# Autodesk Inventor assembly: Manipulator
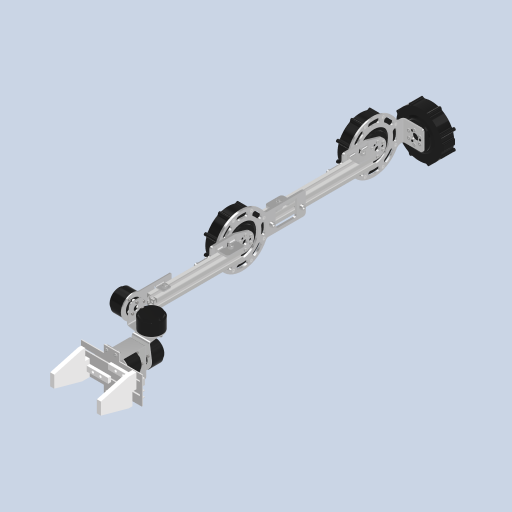
[picture p0: Inventor's stored thumbnail of the model, 512x512]
Saved by Autodesk Inventor 2023 (Build 270158000, 158)
## iProperties
Created: 2024-11-08
Part Number: Manipulator
Document SubType Name: Assembly
Designer: kiyo
Mass: 3708.17 g
Surface Area: 3992.73 cm^2
Volume: 794.407 cm^3
Density: 4.66785 g/cm^3
Author: kiyo
## Documents named in this file (21)
- D:\GitHub\inventor\syu-si\OfficeRobot\Manipulator\Manipulator.iam
- D:\GitHub\inventor\syu-si\OfficeRobot\ReadyMade\Steadywin\GIM8108-8.iam
- D:\GitHub\inventor\syu-si\OfficeRobot\ReadyMade\Steadywin\GIM3505-8_with-driver.ipt
- D:\GitHub\inventor\syu-si\OfficeRobot\Manipulator\wrist-pitch-plate.ipt
- D:\GitHub\inventor\syu-si\OfficeRobot\ReadyMade\Screw\M2-5_6mm.ipt
- D:\GitHub\inventor\syu-si\OfficeRobot\ReadyMade\Screw\CBSH3-8.ipt
- D:\GitHub\inventor\syu-si\OfficeRobot\ReadyMade\Screw\FWSJJ-D5-V2_6-T4_5.ipt
- D:\GitHub\inventor\syu-si\OfficeRobot\ReadyMade\Screw\M2-5_10mm.ipt
- D:\GitHub\inventor\syu-si\OfficeRobot\ReadyMade\Screw\HNTU5-5.ipt
- D:\GitHub\inventor\syu-si\OfficeRobot\Manipulator\sholder_roll_bracket.ipt
- D:\GitHub\inventor\syu-si\OfficeRobot\ReadyMade\Screw\SCB5-8.ipt
- D:\GitHub\inventor\syu-si\OfficeRobot\ReadyMade\Aluminum-frame\NFS5-2020-170-AV15-BV145.ipt
- D:\GitHub\inventor\syu-si\OfficeRobot\Manipulator\wrist_bracket.ipt
- D:\GitHub\inventor\syu-si\OfficeRobot\Hand\Hand.iam
- D:\GitHub\inventor\syu-si\OfficeRobot\ReadyMade\Screw\M2-5_9mm.ipt
- D:\GitHub\inventor\syu-si\OfficeRobot\Manipulator\pitch_plate.ipt
- D:\GitHub\inventor\syu-si\OfficeRobot\ReadyMade\Screw\SCB5-25.ipt
- D:\GitHub\inventor\syu-si\OfficeRobot\ReadyMade\Screw\SCB5-10.ipt
- D:\GitHub\inventor\syu-si\OfficeRobot\Manipulator\elbow-pitch-plate_T4.ipt
- D:\GitHub\inventor\syu-si\OfficeRobot\ReadyMade\Screw\HFBCM3-8.ipt
- D:\GitHub\inventor\syu-si\OfficeRobot\ReadyMade\Aluminum-frame\NFS5-2020-215-AV15-BV180.ipt
## Components (101 placed, 20 different names)
1. sholder_roll_bracket:1 — 挿入:350, 挿入:414, 挿入:493, 挿入:517, 挿入:526, 挿入:527, 挿入:528, 挿入:529, 挿入:530, 挿入:531, 挿入:532, 挿入:533, 挿入:534, 挿入:535, 挿入:536, 挿入:537, 挿入:538, 挿入:539
2. wrist_bracket:2 — 挿入:485, 挿入:552, 挿入:553, 挿入:554
3. wrist_bracket:1
4. wrist-pitch-plate:1 — メイト:71, メイト:72, 正接:48, 正接:49, 角度:76, 角度:77, 角度:78, 正接:50, 正接:51, 挿入:470, 挿入:471, 挿入:494, 挿入:495, 挿入:496
5. NFS5-2020-215-AV15-BV180:1
6. HNTU5-5:32 — 挿入:516
7. SCB5-25:3 — 挿入:516, 正接:83
8. HNTU5-5:33
9. SCB5-10:6 — 正接:84
10. HNTU5-5:34
11. SCB5-10:5 — 正接:85
12. NFS5-2020-170-AV15-BV145:1 — メイト:106, メイト:107, 角度:90, 角度:91, 正接:70, 正接:71, 角度:92, メイト:108, 正接:74, 正接:75, メイト:114, メイト:115
13. M2-5_6mm:16 — 挿入:494
14. M2-5_6mm:17 — 挿入:496
15. M2-5_6mm:18 — 挿入:495
16. Hand:1 [sub-assembly] — 挿入:497, 挿入:501, 挿入:502, 挿入:503, 角度:98, 角度:99
17. M2-5_9mm:1 — 挿入:498, 挿入:503
18. M2-5_9mm:2 — 挿入:500, 挿入:502
19. M2-5_9mm:3 — 挿入:499, 挿入:501
20. HNTU5-5:38
21. SCB5-25:1 — 正接:78
22. HNTU5-5:39
23. SCB5-10:1 — 正接:80
24. HNTU5-5:40
25. SCB5-10:2 — 正接:79
26. HNTU5-5:41 — 角度:90
27. SCB5-10:3 — メイト:106, 正接:70, 正接:82
28. HNTU5-5:42 — 角度:91
29. SCB5-10:4 — メイト:107, 正接:71, 正接:81
30. HNTU5-5:43 — 角度:92
31. SCB5-25:2 — メイト:108, 正接:74, 正接:75, 正接:77
32. pitch_plate:1 — 挿入:512, 正接:78, 正接:79, 正接:80, 角度:96, 挿入:540, 挿入:541, 挿入:542, 挿入:543, 挿入:544, 挿入:545
33. pitch_plate:2 — 挿入:513, メイト:114, メイト:115, 正接:77, 正接:81, 正接:82, 角度:97, 挿入:546, 挿入:547, 挿入:548, 挿入:549, 挿入:550, 挿入:551
34. elbow-pitch-plate_T4:1 — 挿入:514, 挿入:515, 正接:83, 挿入:518, 挿入:519, 挿入:520, 挿入:521, 挿入:522, 挿入:523, 挿入:524, 挿入:525, 正接:84, 正接:85
35. HFBCM3-8:1 — 挿入:521
36. HFBCM3-8:2 — 挿入:524
37. HFBCM3-8:3 — 挿入:525
38. HFBCM3-8:4 — 挿入:523
39. HFBCM3-8:5 — 挿入:522
40. HFBCM3-8:6 — 挿入:518
41. HFBCM3-8:7 — 挿入:519
42. HFBCM3-8:8 — 挿入:520
43. HFBCM3-8:9 — 挿入:531
44. HFBCM3-8:10 — 挿入:532
45. HFBCM3-8:11 — 挿入:530
46. HFBCM3-8:12 — 挿入:529
47. HFBCM3-8:13 — 挿入:528
48. HFBCM3-8:14 — 挿入:533
49. HFBCM3-8:15 — 挿入:526
50. HFBCM3-8:16 — 挿入:527
51. CBSH3-8:1 — 挿入:535
52. CBSH3-8:2 — 挿入:536
53. CBSH3-8:3 — 挿入:538
54. CBSH3-8:4 — 挿入:539
55. CBSH3-8:5 — 挿入:537
56. CBSH3-8:6 — 挿入:534
57. CBSH3-8:7 — 挿入:540
58. CBSH3-8:8 — 挿入:545
59. CBSH3-8:9 — 挿入:548
60. CBSH3-8:10 — 挿入:549
61. CBSH3-8:11 — 挿入:546
62. CBSH3-8:12 — 挿入:541
63. CBSH3-8:13 — 挿入:544
64. CBSH3-8:14 — 挿入:547
65. CBSH3-8:15 — 挿入:551
66. CBSH3-8:16 — 挿入:550
67. CBSH3-8:17 — 挿入:543
68. CBSH3-8:18 — 挿入:542
69. M2-5_6mm:19 — 挿入:552
70. M2-5_6mm:20 — 挿入:553
71. M2-5_6mm:21 — 挿入:554
72. M2-5_6mm:13
73. M2-5_6mm:14
74. M2-5_6mm:15
75. M2-5_10mm:7
76. M2-5_10mm:8
77. M2-5_10mm:9
78. M2-5_10mm:13 — 挿入:453
79. M2-5_10mm:15 — 挿入:454
80. M2-5_10mm:14 — 挿入:455
81. FWSJJ-D5-V2_6-T4_5:16 — 挿入:454
82. FWSJJ-D5-V2_6-T4_5:17 — 挿入:453
83. FWSJJ-D5-V2_6-T4_5:18 — 挿入:455
84. FWSJJ-D5-V2_6-T4_5:10
85. FWSJJ-D5-V2_6-T4_5:11
86. FWSJJ-D5-V2_6-T4_5:12
87. FWSJJ-D5-V2_6-T4_5:13 — 挿入:498
88. FWSJJ-D5-V2_6-T4_5:14 — 挿入:500
89. FWSJJ-D5-V2_6-T4_5:15 — 挿入:499
90. HNTU5-5:22 — 挿入:412, 角度:76
91. SCB5-8:8 — 挿入:412, メイト:72, 正接:49, 正接:50
92. HNTU5-5:23 — 挿入:411, 角度:77
93. SCB5-8:9 — 挿入:411, メイト:71, 正接:48, 正接:51
94. SCB5-25:4
95. HNTU5-5:14 — 角度:78
96. GIM8108-8:1 [sub-assembly] — 挿入:350, 肩ピッチとの角度関係, 環境固定, 環境固定2
97. GIM8108-8:2 [sub-assembly] — 挿入:414, 肩ピッチとの角度関係, 挿入:493, 挿入:512, 角度:96, 挿入:517
98. GIM8108-8:3 [sub-assembly] — 挿入:513, 挿入:514, 挿入:515, 角度:97
99. GIM3505-8_with-driver:9 — 挿入:470, 挿入:471
100. GIM3505-8_with-driver:8 — 挿入:485
101. GIM3505-8_with-driver:10 — 挿入:497
## Relationships (156: Insert 90, Tangent 25, Mate 23, Angle 18)
- 挿入:350 [Insert]: sholder_roll_bracket:1 ↔ GIM8108-8:1
- [Insert] (-3.2 mm): SCB5-25:4 ↔ HNTU5-5:14
- [Insert]: wrist_bracket:1 ↔ M2-5_6mm:13
- [Insert]: wrist_bracket:1 ↔ M2-5_6mm:14
- [Insert]: wrist_bracket:1 ↔ M2-5_6mm:15
- [Insert]: wrist_bracket:1 ↔ GIM3505-8_with-driver:8
- [Insert]: wrist_bracket:1 ↔ GIM3505-8_with-driver:8
- [Insert]: wrist_bracket:1 ↔ M2-5_10mm:7
- [Insert]: wrist_bracket:1 ↔ M2-5_10mm:8
- [Insert]: wrist_bracket:1 ↔ M2-5_10mm:9
- [Insert]: wrist_bracket:1 ↔ FWSJJ-D5-V2_6-T4_5:11
- [Insert]: wrist_bracket:1 ↔ FWSJJ-D5-V2_6-T4_5:12
- [Insert]: wrist_bracket:1 ↔ FWSJJ-D5-V2_6-T4_5:10
- 挿入:411 [Insert] (3.2 mm): HNTU5-5:23 ↔ SCB5-8:9
- 挿入:412 [Insert] (3.2 mm): HNTU5-5:22 ↔ SCB5-8:8
- 挿入:414 [Insert]: sholder_roll_bracket:1 ↔ GIM8108-8:2
- 挿入:453 [Insert] (2 mm): M2-5_10mm:13 ↔ FWSJJ-D5-V2_6-T4_5:17
- 挿入:454 [Insert] (2 mm): M2-5_10mm:15 ↔ FWSJJ-D5-V2_6-T4_5:16
- 挿入:455 [Insert] (2 mm): M2-5_10mm:14 ↔ FWSJJ-D5-V2_6-T4_5:18
- [Insert]: wrist_bracket:2 ↔ M2-5_10mm:13
- [Insert]: wrist_bracket:2 ↔ M2-5_10mm:15
- [Insert]: wrist_bracket:2 ↔ M2-5_10mm:14
- [Insert]: wrist_bracket:2 ↔ GIM3505-8_with-driver:10
- [Insert]: wrist_bracket:2 ↔ GIM3505-8_with-driver:10
- 肩ピッチとの角度関係 [Angle] (0 deg): GIM8108-8:1 ↔ GIM8108-8:2
- 環境固定 [Angle] (-90 deg): GIM8108-8:1
- [Mate]: wrist-pitch-plate:1 ↔ SCB5-25:4
- メイト:71 [Mate]: wrist-pitch-plate:1 ↔ SCB5-8:9
- メイト:72 [Mate]: wrist-pitch-plate:1 ↔ SCB5-8:8
- [Tangent] (0.25 mm): wrist-pitch-plate:1 ↔ SCB5-25:4
- [Tangent] (7.5 mm): wrist-pitch-plate:1 ↔ SCB5-25:4
- 正接:48 [Tangent] (0.25 mm): wrist-pitch-plate:1 ↔ SCB5-8:9
- 正接:49 [Tangent] (0.25 mm): wrist-pitch-plate:1 ↔ SCB5-8:8
- 角度:76 [Angle] (0 deg): wrist-pitch-plate:1 ↔ HNTU5-5:22
- 角度:77 [Angle] (0 deg): wrist-pitch-plate:1 ↔ HNTU5-5:23
- 角度:78 [Angle] (0 deg): wrist-pitch-plate:1 ↔ HNTU5-5:14
- 正接:50 [Tangent] (7.5 mm): wrist-pitch-plate:1 ↔ SCB5-8:8
- 正接:51 [Tangent] (7.5 mm): wrist-pitch-plate:1 ↔ SCB5-8:9
- 挿入:470 [Insert]: wrist-pitch-plate:1 ↔ GIM3505-8_with-driver:9
- 挿入:471 [Insert]: wrist-pitch-plate:1 ↔ GIM3505-8_with-driver:9
- [Mate] (1 mm): NFS5-2020-215-AV15-BV180:1 ↔ HNTU5-5:32
- [Tangent] (32.5 mm): NFS5-2020-215-AV15-BV180:1 ↔ SCB5-25:3
- [Insert] (5.2 mm): HNTU5-5:33 ↔ SCB5-10:6
- [Angle] (0 deg): NFS5-2020-215-AV15-BV180:1 ↔ HNTU5-5:33
- [Mate] (1 mm): NFS5-2020-215-AV15-BV180:1 ↔ HNTU5-5:33
- [Insert] (5.2 mm): HNTU5-5:34 ↔ SCB5-10:5
- [Mate] (1 mm): NFS5-2020-215-AV15-BV180:1 ↔ HNTU5-5:34
- [Mate]: wrist-pitch-plate:1 ↔ NFS5-2020-170-AV15-BV145:1
- [Mate]: wrist-pitch-plate:1 ↔ NFS5-2020-170-AV15-BV145:1
- [Tangent] (22.5 mm): NFS5-2020-170-AV15-BV145:1 ↔ SCB5-25:4
- 挿入:485 [Insert] (4.5 mm): wrist_bracket:2 ↔ GIM3505-8_with-driver:8
- [Insert] (4.5 mm): wrist_bracket:1 ↔ GIM3505-8_with-driver:9
- 環境固定2 [Angle] (0 deg): GIM8108-8:1
- 挿入:493 [Insert]: sholder_roll_bracket:1 ↔ GIM8108-8:2
- 挿入:494 [Insert]: wrist-pitch-plate:1 ↔ M2-5_6mm:16
- 挿入:495 [Insert]: wrist-pitch-plate:1 ↔ M2-5_6mm:18
- 挿入:496 [Insert]: wrist-pitch-plate:1 ↔ M2-5_6mm:17
- 挿入:497 [Insert] (4.5 mm): Hand:1 ↔ GIM3505-8_with-driver:10
- 挿入:498 [Insert] (1.5 mm): M2-5_9mm:1 ↔ FWSJJ-D5-V2_6-T4_5:13
- 挿入:499 [Insert] (1.5 mm): M2-5_9mm:3 ↔ FWSJJ-D5-V2_6-T4_5:15
- 挿入:500 [Insert] (1.5 mm): M2-5_9mm:2 ↔ FWSJJ-D5-V2_6-T4_5:14
- 挿入:501 [Insert]: Hand:1 ↔ M2-5_9mm:3
- 挿入:502 [Insert]: Hand:1 ↔ M2-5_9mm:2
- 挿入:503 [Insert]: Hand:1 ↔ M2-5_9mm:1
- [Insert] (-2.2 mm): HNTU5-5:38 ↔ SCB5-25:1
- [Tangent] (12.5 mm): NFS5-2020-215-AV15-BV180:1 ↔ SCB5-25:1
- [Angle] (0 deg): NFS5-2020-215-AV15-BV180:1 ↔ HNTU5-5:38
- [Insert] (5.2 mm): HNTU5-5:39 ↔ SCB5-10:1
- [Insert] (5.2 mm): HNTU5-5:40 ↔ SCB5-10:2
- [Tangent] (7.5 mm): NFS5-2020-215-AV15-BV180:1 ↔ SCB5-10:2
- [Tangent] (7.5 mm): NFS5-2020-215-AV15-BV180:1 ↔ SCB5-10:1
- [Insert] (5.2 mm): HNTU5-5:41 ↔ SCB5-10:3
- [Insert] (5.2 mm): HNTU5-5:42 ↔ SCB5-10:4
- メイト:106 [Mate] (4 mm): NFS5-2020-170-AV15-BV145:1 ↔ SCB5-10:3
- メイト:107 [Mate] (4 mm): NFS5-2020-170-AV15-BV145:1 ↔ SCB5-10:4
- 角度:90 [Angle] (0 deg): NFS5-2020-170-AV15-BV145:1 ↔ HNTU5-5:41
- 角度:91 [Angle] (0 deg): NFS5-2020-170-AV15-BV145:1 ↔ HNTU5-5:42
- 正接:70 [Tangent] (7.5 mm): NFS5-2020-170-AV15-BV145:1 ↔ SCB5-10:3
- 正接:71 [Tangent] (7.5 mm): NFS5-2020-170-AV15-BV145:1 ↔ SCB5-10:4
- [Insert] (-2.2 mm): HNTU5-5:43 ↔ SCB5-25:2
- 角度:92 [Angle] (0 deg): NFS5-2020-170-AV15-BV145:1 ↔ HNTU5-5:43
- メイト:108 [Mate] (4 mm): NFS5-2020-170-AV15-BV145:1 ↔ SCB5-25:2
- 正接:74 [Tangent] (12.5 mm): NFS5-2020-170-AV15-BV145:1 ↔ SCB5-25:2
- 正接:75 [Tangent] (7.5 mm): NFS5-2020-170-AV15-BV145:1 ↔ SCB5-25:2
- [Mate] (4 mm): NFS5-2020-215-AV15-BV180:1 ↔ SCB5-25:1
- [Tangent] (7.5 mm): NFS5-2020-215-AV15-BV180:1 ↔ SCB5-25:1
- [Mate] (4 mm): NFS5-2020-215-AV15-BV180:1 ↔ SCB5-10:1
- [Mate] (4 mm): NFS5-2020-215-AV15-BV180:1 ↔ SCB5-10:2
- 挿入:512 [Insert]: pitch_plate:1 ↔ GIM8108-8:2
- 挿入:513 [Insert]: pitch_plate:2 ↔ GIM8108-8:3
- [Mate]: NFS5-2020-215-AV15-BV180:1 ↔ pitch_plate:1
- [Mate]: NFS5-2020-215-AV15-BV180:1 ↔ pitch_plate:1
- メイト:114 [Mate]: NFS5-2020-170-AV15-BV145:1 ↔ pitch_plate:2
- メイト:115 [Mate]: NFS5-2020-170-AV15-BV145:1 ↔ pitch_plate:2
- 正接:77 [Tangent] (0.25 mm): SCB5-25:2 ↔ pitch_plate:2
- 正接:78 [Tangent] (0.25 mm): SCB5-25:1 ↔ pitch_plate:1
- [Angle] (0 deg): NFS5-2020-215-AV15-BV180:1 ↔ HNTU5-5:39
- [Angle] (0 deg): NFS5-2020-215-AV15-BV180:1 ↔ HNTU5-5:40
- 正接:79 [Tangent] (0.25 mm): SCB5-10:2 ↔ pitch_plate:1
- 正接:80 [Tangent] (0.25 mm): SCB5-10:1 ↔ pitch_plate:1
- 正接:81 [Tangent] (0.25 mm): SCB5-10:4 ↔ pitch_plate:2
- 正接:82 [Tangent] (0.25 mm): SCB5-10:3 ↔ pitch_plate:2
- 挿入:514 [Insert]: elbow-pitch-plate_T4:1 ↔ GIM8108-8:3
- 挿入:515 [Insert]: elbow-pitch-plate_T4:1 ↔ GIM8108-8:3
- [Angle] (0 deg): NFS5-2020-215-AV15-BV180:1 ↔ HNTU5-5:32
- 挿入:516 [Insert] (-2.2 mm): HNTU5-5:32 ↔ SCB5-25:3
- [Mate] (4 mm): NFS5-2020-215-AV15-BV180:1 ↔ SCB5-25:3
- [Mate]: NFS5-2020-215-AV15-BV180:1 ↔ HNTU5-5:33
- [Mate]: NFS5-2020-215-AV15-BV180:1 ↔ HNTU5-5:34
- [Mate]: NFS5-2020-215-AV15-BV180:1 ↔ elbow-pitch-plate_T4:1
- [Mate]: NFS5-2020-215-AV15-BV180:1 ↔ elbow-pitch-plate_T4:1
- 正接:83 [Tangent] (0.25 mm): SCB5-25:3 ↔ elbow-pitch-plate_T4:1
- 角度:96 [Angle] (0 deg): pitch_plate:1 ↔ GIM8108-8:2
- 角度:97 [Angle] (0 deg): pitch_plate:2 ↔ GIM8108-8:3
- 角度:98 [Angle] (0 deg): Hand:1
- 角度:99 [Angle] (0 deg): Hand:1
- 挿入:517 [Insert]: sholder_roll_bracket:1 ↔ GIM8108-8:2
- 挿入:518 [Insert]: elbow-pitch-plate_T4:1 ↔ HFBCM3-8:6
- 挿入:519 [Insert]: elbow-pitch-plate_T4:1 ↔ HFBCM3-8:7
- 挿入:520 [Insert]: elbow-pitch-plate_T4:1 ↔ HFBCM3-8:8
- 挿入:521 [Insert]: elbow-pitch-plate_T4:1 ↔ HFBCM3-8:1
- 挿入:522 [Insert]: elbow-pitch-plate_T4:1 ↔ HFBCM3-8:5
- 挿入:523 [Insert]: elbow-pitch-plate_T4:1 ↔ HFBCM3-8:4
- 挿入:524 [Insert]: elbow-pitch-plate_T4:1 ↔ HFBCM3-8:2
- 挿入:525 [Insert]: elbow-pitch-plate_T4:1 ↔ HFBCM3-8:3
- 挿入:526 [Insert]: sholder_roll_bracket:1 ↔ HFBCM3-8:15
- 挿入:527 [Insert]: sholder_roll_bracket:1 ↔ HFBCM3-8:16
- 挿入:528 [Insert]: sholder_roll_bracket:1 ↔ HFBCM3-8:13
- 挿入:529 [Insert]: sholder_roll_bracket:1 ↔ HFBCM3-8:12
- 挿入:530 [Insert]: sholder_roll_bracket:1 ↔ HFBCM3-8:11
- 挿入:531 [Insert]: sholder_roll_bracket:1 ↔ HFBCM3-8:9
- 挿入:532 [Insert]: sholder_roll_bracket:1 ↔ HFBCM3-8:10
- 挿入:533 [Insert]: sholder_roll_bracket:1 ↔ HFBCM3-8:14
- 挿入:534 [Insert]: sholder_roll_bracket:1 ↔ CBSH3-8:6
- 挿入:535 [Insert]: sholder_roll_bracket:1 ↔ CBSH3-8:1
- 挿入:536 [Insert]: sholder_roll_bracket:1 ↔ CBSH3-8:2
- 挿入:537 [Insert]: sholder_roll_bracket:1 ↔ CBSH3-8:5
- 挿入:538 [Insert]: sholder_roll_bracket:1 ↔ CBSH3-8:3
- 挿入:539 [Insert]: sholder_roll_bracket:1 ↔ CBSH3-8:4
- 挿入:540 [Insert]: pitch_plate:1 ↔ CBSH3-8:7
- 挿入:541 [Insert]: pitch_plate:1 ↔ CBSH3-8:12
- 挿入:542 [Insert]: pitch_plate:1 ↔ CBSH3-8:18
- 挿入:543 [Insert]: pitch_plate:1 ↔ CBSH3-8:17
- 挿入:544 [Insert]: pitch_plate:1 ↔ CBSH3-8:13
- 挿入:545 [Insert]: pitch_plate:1 ↔ CBSH3-8:8
- 挿入:546 [Insert]: pitch_plate:2 ↔ CBSH3-8:11
- 挿入:547 [Insert]: pitch_plate:2 ↔ CBSH3-8:14
- 挿入:548 [Insert]: pitch_plate:2 ↔ CBSH3-8:9
- 挿入:549 [Insert]: pitch_plate:2 ↔ CBSH3-8:10
- 挿入:550 [Insert]: pitch_plate:2 ↔ CBSH3-8:16
- 挿入:551 [Insert]: pitch_plate:2 ↔ CBSH3-8:15
- 正接:84 [Tangent] (0.25 mm): SCB5-10:6 ↔ elbow-pitch-plate_T4:1
- 正接:85 [Tangent] (0.25 mm): SCB5-10:5 ↔ elbow-pitch-plate_T4:1
- 挿入:552 [Insert]: wrist_bracket:2 ↔ M2-5_6mm:19
- 挿入:553 [Insert]: wrist_bracket:2 ↔ M2-5_6mm:20
- 挿入:554 [Insert]: wrist_bracket:2 ↔ M2-5_6mm:21
## Named parameters: d516_d512 = 0 mm, d517_d513 = 0 mm, d519_d268 = 0 mm, d520_d269 = 0 mm, d521_d270 = 0 mm, d782_d733_d492_d466 = 5.2 mm, d787_d782_d733_d492_d466 = 5.2 mm, d14_d733_d492_d466 = 5.2 mm, d880_d14_d733_d492_d466 = 5.2 mm, d889_d14_d733_d492_d466 = 5.2 mm, d890_d14_d733_d492_d466 = 5.2 mm, d900_d25 = -2.2 mm
